# Autodesk Inventor assembly: Body 2.0
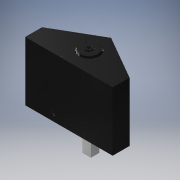
[picture p0: Inventor's stored thumbnail of the model, 180x180]
Saved by Autodesk Inventor 2017 (Build 210142000, 142)
## iProperties
Created: 2019-05-22
Part Number: Body 2.0
Document SubType Name: Assembly
Designer: Dell
Mass: 8839.43 g
Surface Area: 20740.7 cm^2
Volume: 10189.8 cm^3
Density: 0.867479 g/cm^3
Author: Dell
## Documents named in this file (12)
- C:\Users\Dell\Documents\GitHub\tr2\Body 2.0\Body 2.0.iam
- C:\Users\Dell\Documents\GitHub\tr2\Body 2.0\BA01.ipt
- C:\Users\Dell\Documents\GitHub\tr2\Body 2.0\BA02.ipt
- C:\Users\Dell\Documents\GitHub\tr2\Body 2.0\BA03.ipt
- C:\Users\Dell\Documents\GitHub\tr2\Body 2.0\BA04.ipt
- C:\Users\Dell\Documents\GitHub\tr2\Body 2.0\BA05.ipt
- C:\Users\Dell\Documents\GitHub\tr2\Body 2.0\BA06.ipt
- C:\Users\Dell\Documents\GitHub\tr2\Body 2.0\BA07.ipt
- C:\Users\Dell\Documents\GitHub\tr2\Body 2.0\BA08.ipt
- C:\Users\Dell\Documents\GitHub\tr2\Body 2.0\ST01.ipt
- C:\Users\Dell\Documents\GitHub\tr2\Actuator 1.3\Actuator 1.3.iam
- C:\Users\Dell\Documents\GitHub\tr2\Body 2.0\AE01.ipt
## Components (14 placed, 11 different names)
1. BA01:1 — Mate:1, Flush:1, Flush:2, Mate:2, Flush:3, Flush:4, Mate:4, Mate:6, Flush:5, Mate:8, Mate:10
2. BA02:1 — Mate:1, Flush:1, Flush:2, Mate:3, Mate:9, Mate:13, Mate:14
3. BA03:1 — Mate:2, Mate:3, Flush:3, Mate:5, Mate:15, Mate:16
4. BA04:1 — Flush:4, Mate:4, Mate:5, Mate:7
5. BA05:1 — Mate:6, Flush:5, Mate:7
6. BA06:1 — Mate:8, Mate:9, Mate:10, Mate:11, Mate:12
7. BA07:1 — Mate:11, Mate:12, Mate:13, Mate:26, Mate:27, Flush:9, Flush:10, Mate:28, Mate:29, Mate:30
8. BA08:1 — Mate:14, Mate:15, Mate:16, Mate:17, Mate:18, Flush:6, Mate:19, Mate:20, Flush:7, Mate:21, Mate:22, Flush:8, Mate:23, Mate:24, Mate:25
9. ST01:1 — Mate:17, Mate:18, Flush:6
10. ST01:2 — Mate:19, Mate:20, Flush:7
11. ST01:3 — Mate:21, Mate:22, Flush:8
12. Actuator 1.3:1 [sub-assembly] — Mate:23, Mate:24, Mate:25
13. AE01:1 — Mate:27, Flush:9, Mate:29
14. AE01:2 — Mate:26, Flush:10, Mate:28, Mate:30
## Relationships (40: Mate 30, Flush 10)
- Mate:1: BA01:1 ↔ BA02:1
- Flush:1: BA01:1 ↔ BA02:1
- Flush:2: BA01:1 ↔ BA02:1
- Mate:2: BA01:1 ↔ BA03:1
- Mate:3: BA02:1 ↔ BA03:1
- Flush:3: BA01:1 ↔ BA03:1
- Flush:4: BA01:1 ↔ BA04:1
- Mate:4: BA01:1 ↔ BA04:1
- Mate:5: BA03:1 ↔ BA04:1
- Mate:6: BA01:1 ↔ BA05:1
- Flush:5: BA01:1 ↔ BA05:1
- Mate:7: BA04:1 ↔ BA05:1
- Mate:8: BA01:1 ↔ BA06:1
- Mate:9: BA02:1 ↔ BA06:1
- Mate:10: BA01:1 ↔ BA06:1
- Mate:11: BA06:1 ↔ BA07:1
- Mate:12: BA06:1 ↔ BA07:1
- Mate:13: BA02:1 ↔ BA07:1
- Mate:14: BA02:1 ↔ BA08:1
- Mate:15: BA03:1 ↔ BA08:1
- Mate:16: BA03:1 ↔ BA08:1
- Mate:17: BA08:1 ↔ ST01:1
- Mate:18: BA08:1 ↔ ST01:1
- Flush:6: BA08:1 ↔ ST01:1
- Mate:19: BA08:1 ↔ ST01:2
- Mate:20: BA08:1 ↔ ST01:2
- Flush:7: BA08:1 ↔ ST01:2
- Mate:21: BA08:1 ↔ ST01:3
- Mate:22: BA08:1 ↔ ST01:3
- Flush:8: BA08:1 ↔ ST01:3
- Mate:23: BA08:1 ↔ Actuator 1.3:1
- Mate:24: BA08:1 ↔ Actuator 1.3:1
- Mate:25: BA08:1 ↔ Actuator 1.3:1
- Mate:26: BA07:1 ↔ AE01:2
- Mate:27: BA07:1 ↔ AE01:1
- Flush:9: BA07:1 ↔ AE01:1
- Flush:10: BA07:1 ↔ AE01:2
- Mate:28: BA07:1 ↔ AE01:2
- Mate:29: BA07:1 ↔ AE01:1
- Mate:30: BA07:1 ↔ AE01:2
